# Autodesk Inventor assembly: CamMountOnly
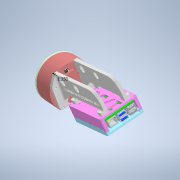
[picture p0: Inventor's stored thumbnail of the model, 180x180]
Saved by Autodesk Inventor 2020 (Build 240168000, 168)
## iProperties
Created: 2020-02-08
Part Number: CamMountOnly
Document SubType Name: Assembly
Designer: Chris Gerth
Author: Chris Gerth
## Documents named in this file (10)
- C:\Users\Chris Gerth\Documents\Robotics\RobotCasserole2020\piVisionCase\CamMountOnly.iam
- C:\Users\Chris Gerth\Documents\Robotics\RobotCasserole2020\piVisionCase\cameraToChurroSplineRight.ipt
- C:\Users\Chris Gerth\Documents\Robotics\RobotCasserole2020\piVisionCase\cameraToChurroSplineLeft.ipt
- C:\Users\Chris Gerth\Documents\Robotics\RobotCasserole2020\piVisionCase\camHolderTop.ipt
- C:\Users\Chris Gerth\Documents\Robotics\RobotCasserole2020\piVisionCase\camHolderBottom.ipt
- C:\Users\Chris Gerth\Documents\Robotics\RobotCasserole2020\piVisionCase\camera.ipt
- C:\Users\Chris Gerth\Documents\Robotics\RobotCasserole2020\piVisionCase\ledRing.ipt
- C:\Users\Chris Gerth\Documents\Robotics\RobotCasserole2020\piVisionCase\piBottom.ipt
- C:\Users\Chris Gerth\Documents\Robotics\RobotCasserole2020\piVisionCase\Raspberry Pi 4 Model B.iam
- C:\Users\Chris Gerth\Documents\Robotics\RobotCasserole2020\piVisionCase\piTop.ipt
## Components (9 placed, 9 different names)
1. cameraToChurroSplineRight:1 — Mate:19, Mate:22, Mate:24, Mate:31
2. cameraToChurroSplineLeft:1 — Mate:11, Mate:23, Mate:25, Mate:30
3. camHolderTop:1 — Mate:17, Mate:18, Mate:19, Mate:20
4. camHolderBottom:1 — Mate:11, Mate:14, Mate:15, Mate:16, Mate:17, Mate:18, Mate:22
5. camera:1 — Mate:14, Mate:15, Mate:16, Mate:21
6. ledRing:1 — Mate:20, Mate:21
7. piBottom:1 — Mate:23, Mate:24, Mate:25, Mate:26, Mate:27, Mate:28, Mate:29, Flush:3, Flush:4, Mate:30, Mate:31
8. Raspberry Pi 4 Model B:1 [sub-assembly] — Mate:26, Mate:27, Mate:28
9. piTop:1 — Mate:29, Flush:3, Flush:4
## Relationships (21: Mate 19, Flush 2)
- Mate:11: cameraToChurroSplineLeft:1 ↔ camHolderBottom:1
- Mate:14: camHolderBottom:1 ↔ camera:1
- Mate:15: camHolderBottom:1 ↔ camera:1
- Mate:16: camHolderBottom:1 ↔ camera:1
- Mate:17: camHolderTop:1 ↔ camHolderBottom:1
- Mate:18: camHolderTop:1 ↔ camHolderBottom:1
- Mate:19: cameraToChurroSplineRight:1 ↔ camHolderTop:1
- Mate:20: camHolderTop:1 ↔ ledRing:1
- Mate:21: camera:1 ↔ ledRing:1
- Mate:22: cameraToChurroSplineRight:1 ↔ camHolderBottom:1
- Mate:23: cameraToChurroSplineLeft:1 ↔ piBottom:1
- Mate:24: cameraToChurroSplineRight:1 ↔ piBottom:1
- Mate:25: cameraToChurroSplineLeft:1 ↔ piBottom:1
- Mate:26: piBottom:1 ↔ Raspberry Pi 4 Model B:1
- Mate:27 (3.175 mm): piBottom:1 ↔ Raspberry Pi 4 Model B:1
- Mate:28: piBottom:1 ↔ Raspberry Pi 4 Model B:1
- Mate:29: piBottom:1 ↔ piTop:1
- Flush:3: piBottom:1 ↔ piTop:1
- Flush:4: piBottom:1 ↔ piTop:1
- Mate:30: cameraToChurroSplineLeft:1 ↔ piBottom:1
- Mate:31: cameraToChurroSplineRight:1 ↔ piBottom:1
